# Autodesk Inventor assembly: assembled-feed
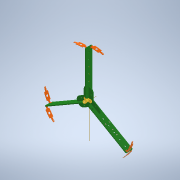
[picture p0: Inventor's stored thumbnail of the model, 180x180]
Saved by Autodesk Inventor 2021 (Build 250183000, 183)
## iProperties
Created: 2020-09-03
Part Number: assembled-feed
Document SubType Name: Assembly
Designer: dsouthall
Author: dsouthall
## Documents named in this file (3)
- C:\Users\dsouthall\OneDrive - The University of Chicago\Hpol\Model 8 in\assembled-feed.iam
- C:\Users\dsouthall\OneDrive - The University of Chicago\Hpol\Model 8 in\source\hub\tri-slot-hub.iam
- C:\Users\dsouthall\OneDrive - The University of Chicago\Hpol\Model 8 in\assembled-feed_feedline_8in.iam
## Components (4 placed, 2 different names)
1. tri-slot-hub:1 [sub-assembly] — Mate:10, Angle:1, Mate:17, Mate:20, Mate:21, Mate:22, Mate:23, Mate:24, Mate:25, Mate:26, Mate:27, Mate:28, Mate:29, Mate:30
2. assembled-feed_feedline_8in:1 [sub-assembly] — Mate:21, Mate:22, Mate:23
3. assembled-feed_feedline_8in:2 [sub-assembly] — Mate:24, Mate:25, Mate:26
4. assembled-feed_feedline_8in:3 [sub-assembly] — Mate:27, Mate:28, Mate:29
## Relationships (15: Mate 13, Angle 1, Flush 1)
- Mate:10: tri-slot-hub:1
- Angle:1 (0 deg): tri-slot-hub:1
- Mate:17: tri-slot-hub:1
- Mate:20: tri-slot-hub:1
- Flush:1 (-3.9973 mm)
- Mate:21: tri-slot-hub:1 ↔ assembled-feed_feedline_8in:1
- Mate:22: tri-slot-hub:1 ↔ assembled-feed_feedline_8in:1
- Mate:23: tri-slot-hub:1 ↔ assembled-feed_feedline_8in:1
- Mate:24: tri-slot-hub:1 ↔ assembled-feed_feedline_8in:2
- Mate:25: tri-slot-hub:1 ↔ assembled-feed_feedline_8in:2
- Mate:26: tri-slot-hub:1 ↔ assembled-feed_feedline_8in:2
- Mate:27: tri-slot-hub:1 ↔ assembled-feed_feedline_8in:3
- Mate:28: tri-slot-hub:1 ↔ assembled-feed_feedline_8in:3
- Mate:29: tri-slot-hub:1 ↔ assembled-feed_feedline_8in:3
- Mate:30 (-0.8 mm): tri-slot-hub:1
